# Autodesk Inventor assembly: Assembly 3D Cutting
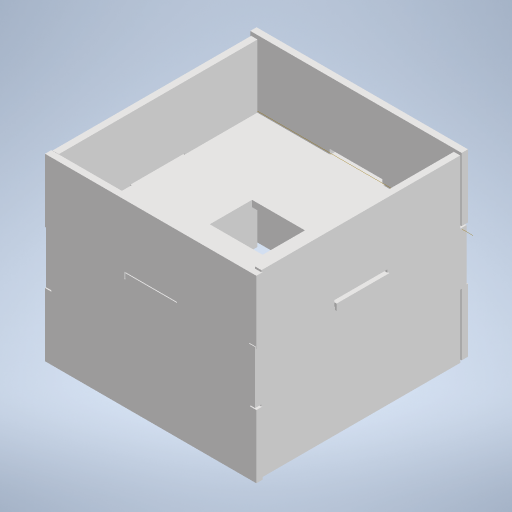
[picture p0: Inventor's stored thumbnail of the model, 512x512]
Saved by Autodesk Inventor 2023 (Build 270158000, 158)
## iProperties
Created: 2023-02-07
Part Number: Assembly 3D Cutting
Document SubType Name: Assembly
Designer: Asus
Author: Asus
## Documents named in this file (4)
- D:\Eksintek\Pneumatik SKUBI Sby\3D Cutting\Kotak Taruh Selesai\End_Assembly 3D Cutting.iam
- D:\Eksintek\Pneumatik SKUBI Sby\3D Cutting\Kotak Taruh Selesai\End_Samping.ipt
- D:\Eksintek\Pneumatik SKUBI Sby\3D Cutting\Kotak Taruh Selesai\End_Depan.ipt
- D:\Eksintek\Pneumatik SKUBI Sby\3D Cutting\Kotak Taruh Selesai\End_bolongan.ipt
## Components (5 placed, 3 different names)
1. End_Samping:1
2. End_Depan:1
3. End_Depan:2
4. End_Samping:2 — Mate:2
5. End_bolongan:1 — Mate:1
## Relationships (2: Mate 2)
- Mate:1: End_bolongan:1
- Mate:2: End_Samping:2
